# Autodesk Inventor assembly: Carriage
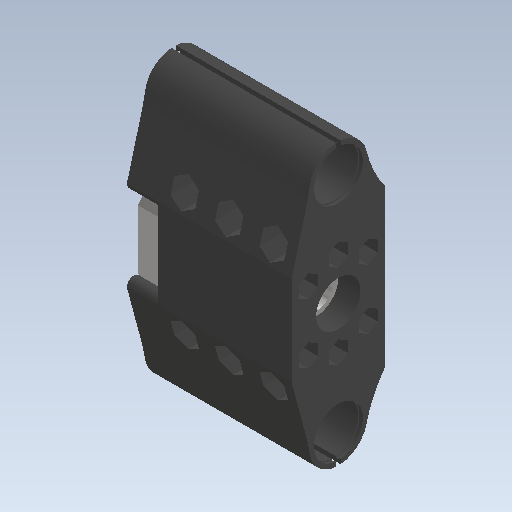
[picture p0: Inventor's stored thumbnail of the model, 512x512]
Saved by Autodesk Inventor 2020 (Build 240168000, 168)
## iProperties
Created: 2022-03-31
Part Number: Carriage
Document SubType Name: Assembly
Designer: mikoma
Mass: 386.466 g
Surface Area: 674.096 cm^2
Volume: 203.129 cm^3
Density: 1.90257 g/cm^3
Author: mikoma
## Documents named in this file (3)
- D:\KONIECTEGOKOŁCHOZU\MGR\model\Workspaces\Obszar roboczy\assembly_v3\C\Carriage.iam
- D:\KONIECTEGOKOŁCHOZU\MGR\model\Workspaces\Obszar roboczy\assembly_OLD\złożenie\Cartesian1_XYCarriage.ipt
- D:\KONIECTEGOKOŁCHOZU\MGR\model\Workspaces\Obszar roboczy\content\manipulatorSharedParts\Cartesian1_BallNut.ipt
## Components (2 placed, 2 different names)
1. Cartesian1_XYCarriage:1 — Zestawiające:1, Równoległe:1, Zestawiające:2, Zestawiające:3, Zestawiające:4, Zestawiające:5
2. Cartesian1_BallNut:1 — Zestawiające:3, Zestawiające:4, Zestawiające:5
## Relationships (6: Mate 5, Flush 1)
- Zestawiające:1 [Mate]: Cartesian1_XYCarriage:1
- Równoległe:1 [Flush]: Cartesian1_XYCarriage:1
- Zestawiające:2 [Mate]: Cartesian1_XYCarriage:1
- Zestawiające:3 [Mate]: Cartesian1_XYCarriage:1 ↔ Cartesian1_BallNut:1
- Zestawiające:4 [Mate]: Cartesian1_XYCarriage:1 ↔ Cartesian1_BallNut:1
- Zestawiające:5 [Mate]: Cartesian1_XYCarriage:1 ↔ Cartesian1_BallNut:1
